# Autodesk Inventor assembly: ABME-2020-4-R
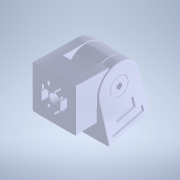
[picture p0: Inventor's stored thumbnail of the model, 180x180]
Saved by Autodesk Inventor 2021.1 (Build 251245010, 245A)
## iProperties
Created: 2018-09-13
Part Number: ABME-2020-4-R
Description: STEP AP214
Document SubType Name: Assembly
Designer: gisen
Sending System: SolidWorks 2018
Preprocessor: SwSTEP 2.0
Title: ABME-2020-4-R.STEP
Revision Number: ANY
## Documents named in this file (5)
- C:\Users\gisen\GitProjects\CAD-Data\GeneralComponentsTemplate\Fittings\BasicFrameMultiEndConnectorR.iam
- C:\Users\gisen\GitProjects\CAD-Data\GeneralComponentsTemplate\Fittings\BasicFrameMultiEndConnectorR\ABME-2020-4-R.ipt
- C:\Users\gisen\GitProjects\CAD-Data\GeneralComponentsTemplate\Fittings\BasicFrameMultiEndConnectorR\ABME-2020-4-R-2.ipt
- C:\Users\gisen\GitProjects\CAD-Data\GeneralComponentsTemplate\Fittings\BasicFrameMultiEndConnectorR\ABME-2020-4-R-1.ipt
- C:\Users\gisen\GitProjects\CAD-Data\GeneralComponentsTemplate\Fittings\BasicFrameMultiEndConnectorR\ABME-2020-4-R-4.ipt
## Components (7 placed, 7 different names)
1. ABME-2020-4-R_1 — メイト:1, メイト:2, フラッシュ:2, メイト:15
2. ABME-2020-4-R_2 — メイト:1, メイト:2, メイト:10, メイト:12
3. ABME-2020-4-R_3
4. ABME-2020-4-R_4 — フラッシュ:1, メイト:3, メイト:10
5. ABME-2020-4-R_5
6. FCS-04_ÃÞÌ«ÙÄ L8_8 — フラッシュ:1, メイト:3, メイト:12
7. FCS-04_ÃÞÌ«ÙÄ L8_9 — フラッシュ:2, メイト:15
## Relationships (8: Mate 6, Flush 2)
- メイト:1 [Mate]: ABME-2020-4-R_1 ↔ ABME-2020-4-R_2
- メイト:2 [Mate]: ABME-2020-4-R_1 ↔ ABME-2020-4-R_2
- フラッシュ:1 [Flush]: ABME-2020-4-R_4 ↔ FCS-04_ÃÞÌ«ÙÄ L8_8
- メイト:3 [Mate]: ABME-2020-4-R_4 ↔ FCS-04_ÃÞÌ«ÙÄ L8_8
- メイト:10 [Mate]: ABME-2020-4-R_2 ↔ ABME-2020-4-R_4
- メイト:12 [Mate]: ABME-2020-4-R_2 ↔ FCS-04_ÃÞÌ«ÙÄ L8_8
- フラッシュ:2 [Flush]: ABME-2020-4-R_1 ↔ FCS-04_ÃÞÌ«ÙÄ L8_9
- メイト:15 [Mate]: ABME-2020-4-R_1 ↔ FCS-04_ÃÞÌ«ÙÄ L8_9
